# Autodesk Inventor assembly: fc18_010
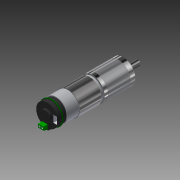
[picture p0: Inventor's stored thumbnail of the model, 180x180]
Saved by Autodesk Inventor 2018 (Build 220112000, 112)
## iProperties
Category: Motors
Company: Autodesk Inc.
Created: 2017-11-21
Part Number: fc18_010
Document SubType Name: Assembly
Designer: Autodesk Inc.
Catalog Web Link: http://firstchoicebyandymark.com/fc18-010
Vendor: AndyMark Inc.
Author: Autodesk Inc.
Keywords: FIRSTChoice
## Documents named in this file (3)
- F:\FIRST 2018\FIRST 2018 FirstChoice\fc18-010_GearMotorEncoder.iam
- F:\FIRST 2018\FIRST 2018 FirstChoice\Parts\fc17-017_GearMotor.ipt
- F:\FIRST 2018\FIRST 2018 FirstChoice\Parts\Hall Effect Encoder for PG Gearboxes.ipt
## Components (2 placed, 2 different names)
1. fc17-017_GearMotor:1 — Insert:1, Angle:1
2. Hall Effect Encoder for PG Gearboxes:1 — Insert:1, Angle:1
## Relationships (2: Insert 1, Angle 1)
- Insert:1: fc17-017_GearMotor:1 ↔ Hall Effect Encoder for PG Gearboxes:1
- Angle:1 (0 deg): fc17-017_GearMotor:1 ↔ Hall Effect Encoder for PG Gearboxes:1
